# Autodesk Inventor assembly: chest_cover
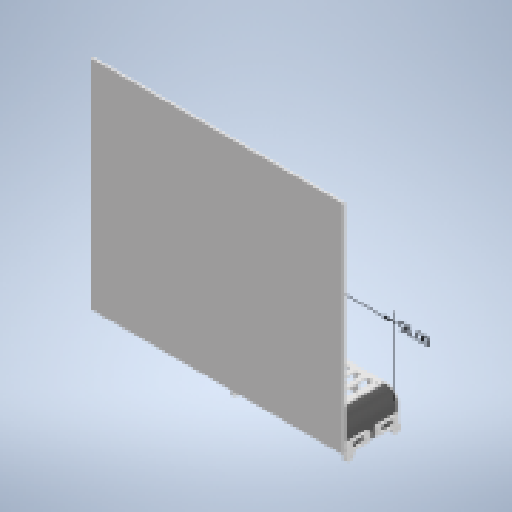
[picture p0: Inventor's stored thumbnail of the model, 512x512]
Saved by Autodesk Inventor 2024.1 (Build 281209000, 209)
## iProperties
Created: 2024-02-14
Part Number: chest_cover
Document SubType Name: Assembly
Designer: hibik
Author: hibik
## Documents named in this file (6)
- C:\Users\hibik\Desktop\ロボメカ\HR\2024.02.11 Rl\02.11 ProtType\chest_cover.iam
- C:\Users\hibik\Desktop\ロボメカ\HR\2024.02.11 Rl\02.11 ProtType\chest_cover_top.ipt
- C:\Users\hibik\Desktop\ロボメカ\HR\2024.02.11 Rl\02.11 ProtType\chest_cover_side.ipt
- C:\Users\hibik\Desktop\ロボメカ\HR\2024.02.11 Rl\02.11 ProtType\chest_cover_side_joint.ipt
- C:\Users\hibik\Desktop\ロボメカ\HR\2024.02.11 Rl\02.11 ProtType\chest_cover_upun.ipt
- C:\Users\hibik\Desktop\ロボメカ\HR\2024.02.11 Rl\02.11 ProtType\chest_cover_upper.ipt
## Components (8 placed, 5 different names)
1. chest_cover_top:1 — 挿入:1, 挿入:2
2. chest_cover_side:1 — 挿入:1, 挿入:2, メイト:1, フラッシュ:1, フラッシュ:2, メイト:2, フラッシュ:3, フラッシュ:4, メイト:3, フラッシュ:5, フラッシュ:6, 挿入:3, 挿入:4, 挿入:5, 挿入:6, メイト:4, フラッシュ:7, フラッシュ:8
3. chest_cover_side_joint:1 — メイト:2, フラッシュ:3, フラッシュ:4
4. chest_cover_side_joint:2 — メイト:1, フラッシュ:1, フラッシュ:2
5. chest_cover_upun:1 — メイト:3, フラッシュ:5, フラッシュ:6
6. chest_cover_side_joint:3 — 挿入:3, 挿入:4
7. chest_cover_side_joint:4 — 挿入:5, 挿入:6
8. chest_cover_upper:1 — メイト:4, フラッシュ:7, フラッシュ:8
## Relationships (18: Flush 8, Insert 6, Mate 4)
- 挿入:1 [Insert]: chest_cover_top:1 ↔ chest_cover_side:1
- 挿入:2 [Insert]: chest_cover_top:1 ↔ chest_cover_side:1
- メイト:1 [Mate]: chest_cover_side:1 ↔ chest_cover_side_joint:2
- フラッシュ:1 [Flush]: chest_cover_side:1 ↔ chest_cover_side_joint:2
- フラッシュ:2 [Flush]: chest_cover_side:1 ↔ chest_cover_side_joint:2
- メイト:2 [Mate]: chest_cover_side:1 ↔ chest_cover_side_joint:1
- フラッシュ:3 [Flush]: chest_cover_side:1 ↔ chest_cover_side_joint:1
- フラッシュ:4 [Flush]: chest_cover_side:1 ↔ chest_cover_side_joint:1
- メイト:3 [Mate]: chest_cover_side:1 ↔ chest_cover_upun:1
- フラッシュ:5 [Flush]: chest_cover_side:1 ↔ chest_cover_upun:1
- フラッシュ:6 [Flush]: chest_cover_side:1 ↔ chest_cover_upun:1
- 挿入:3 [Insert]: chest_cover_side:1 ↔ chest_cover_side_joint:3
- 挿入:4 [Insert]: chest_cover_side:1 ↔ chest_cover_side_joint:3
- 挿入:5 [Insert]: chest_cover_side:1 ↔ chest_cover_side_joint:4
- 挿入:6 [Insert]: chest_cover_side:1 ↔ chest_cover_side_joint:4
- メイト:4 [Mate]: chest_cover_side:1 ↔ chest_cover_upper:1
- フラッシュ:7 [Flush]: chest_cover_side:1 ↔ chest_cover_upper:1
- フラッシュ:8 [Flush]: chest_cover_side:1 ↔ chest_cover_upper:1
